# Autodesk Inventor assembly: left
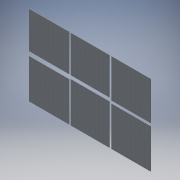
[picture p0: Inventor's stored thumbnail of the model, 180x180]
Saved by Autodesk Inventor 2019 (Build 230136000, 136)
## iProperties
Created: 2018-07-10
Part Number: left
Document SubType Name: Assembly
Designer: User
Author: User
## Documents named in this file (7)
- C:\Users\User\Desktop\Room Model\left.iam
- C:\Users\User\Desktop\Room Model\left_0_0.ipt
- C:\Users\User\Desktop\Room Model\left_0_1.ipt
- C:\Users\User\Desktop\Room Model\left_0_2.ipt
- C:\Users\User\Desktop\Room Model\left_1_1.ipt
- C:\Users\User\Desktop\Room Model\left_1_2.ipt
- C:\Users\User\Desktop\Room Model\left_1_0.ipt
## Components (6 placed, 6 different names)
1. left_0_0:1 — Rigid:1, Rigid:5
2. left_0_1:1 — Rigid:1, Rigid:2
3. left_0_2:1 — Rigid:2
4. left_1_0:1 — Rigid:3, Rigid:5
5. left_1_1:2 — Rigid:3, Rigid:4
6. left_1_2:1 — Rigid:4
## Relationships (5: WeldJoint 5)
- Rigid:1 [WeldJoint] (53.975 mm): left_0_0:1 ↔ left_0_1:1
- Rigid:2 [WeldJoint] (63.5 mm): left_0_1:1 ↔ left_0_2:1
- Rigid:3 [WeldJoint] (53.975 mm): left_1_0:1 ↔ left_1_1:2
- Rigid:4 [WeldJoint] (63.5 mm): left_1_1:2 ↔ left_1_2:1
- Rigid:5 [WeldJoint] (127 mm): left_0_0:1 ↔ left_1_0:1
